# Autodesk Inventor assembly: Lift.04.00.00.00
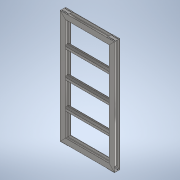
[picture p0: Inventor's stored thumbnail of the model, 180x180]
Saved by Autodesk Inventor 2021 (Build 250183000, 183)
## iProperties
_SolveAssemblyDoc: Frame Generator Solve Assembly
_Version: 25.0.0
Created: 2020-09-20
Part Number: Lift.04.00.00.00
Document SubType Name: Assembly
Designer: Kostya
Author: Kostya
## Documents named in this file (4)
- C:\Lift\Lift.04.00.00.00.iam
- C:\Lift\Lift.04.00.00.02.ipt
- C:\Lift\Lift.04.00.00.00\Frame\Frame 1600625129294.iam
- C:\Lift\Lift.04.00.00.01.ipt
## Components (6 placed, 3 different names)
1. Lift.04.00.00.02:1
2. Frame 1600625129294:1 [sub-assembly] — Совмещение:1, Заподлицо:1, Заподлицо:2, Совмещение:2, Заподлицо:3, Заподлицо:4, Совмещение:3, Заподлицо:5, Заподлицо:6, Заподлицо:7, Заподлицо:8, Совмещение:4
3. Lift.04.00.00.01:1 — Совмещение:1, Заподлицо:1, Заподлицо:2
4. Lift.04.00.00.01:2 — Совмещение:2, Заподлицо:3, Заподлицо:4
5. Lift.04.00.00.01:3 — Заподлицо:7, Заподлицо:8, Совмещение:4
6. Lift.04.00.00.01:4 — Совмещение:3, Заподлицо:5, Заподлицо:6
## Relationships (12: Flush 8, Mate 4)
- Совмещение:1 [Mate]: Frame 1600625129294:1 ↔ Lift.04.00.00.01:1
- Заподлицо:1 [Flush]: Frame 1600625129294:1 ↔ Lift.04.00.00.01:1
- Заподлицо:2 [Flush]: Frame 1600625129294:1 ↔ Lift.04.00.00.01:1
- Совмещение:2 [Mate]: Frame 1600625129294:1 ↔ Lift.04.00.00.01:2
- Заподлицо:3 [Flush]: Frame 1600625129294:1 ↔ Lift.04.00.00.01:2
- Заподлицо:4 [Flush]: Frame 1600625129294:1 ↔ Lift.04.00.00.01:2
- Совмещение:3 [Mate]: Frame 1600625129294:1 ↔ Lift.04.00.00.01:4
- Заподлицо:5 [Flush]: Frame 1600625129294:1 ↔ Lift.04.00.00.01:4
- Заподлицо:6 [Flush]: Frame 1600625129294:1 ↔ Lift.04.00.00.01:4
- Заподлицо:7 [Flush]: Frame 1600625129294:1 ↔ Lift.04.00.00.01:3
- Заподлицо:8 [Flush]: Frame 1600625129294:1 ↔ Lift.04.00.00.01:3
- Совмещение:4 [Mate]: Frame 1600625129294:1 ↔ Lift.04.00.00.01:3
